# Autodesk Inventor assembly: Assembly
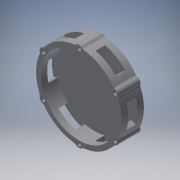
[picture p0: Inventor's stored thumbnail of the model, 180x180]
Saved by Autodesk Inventor 2018 (Build 220112000, 112)
## iProperties
Created: 2018-01-25
Part Number: Assembly
Document SubType Name: Assembly
Designer: Rus
Author: Rus
## Documents named in this file (3)
- C:\Users\Rus\Documents\3D Models\Siren\Assembly.iam
- C:\Users\Rus\Documents\3D Models\Siren\Slotted Case 1.ipt
- C:\Users\Rus\Documents\3D Models\Siren\Impeller 1.ipt
## Components (2 placed, 2 different names)
1. Slotted Case 1:1 — Insert:1
2. Impeller 1:1 — Insert:1
## Relationships (1: Insert 1)
- Insert:1: Slotted Case 1:1 ↔ Impeller 1:1
